# Autodesk Inventor assembly: Assembly_Cube_FluorescenceFilterSlider
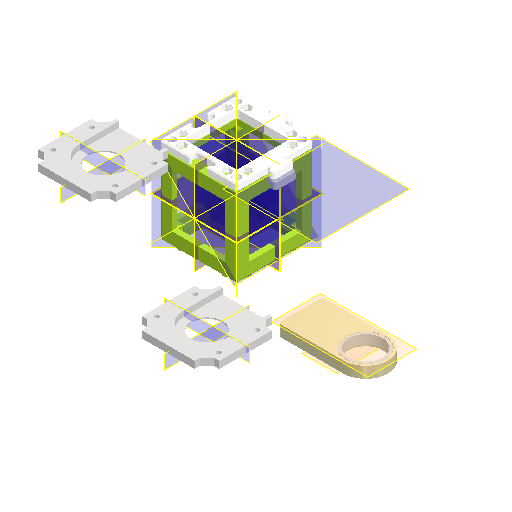
[picture p0: Inventor's stored thumbnail of the model, 512x512]
Saved by Autodesk Inventor 2025.1 (Build 291241020, 241B)
## iProperties
Created: 2023-11-21
Part Number: Assembly_Cube_FluorescenceFilterSlider
Document SubType Name: Assembly
Designer: diederichbenedict
Author: diederichbenedict
## Documents named in this file (5)
- C:\Users\diederichbenedict\Dropbox\Dokumente\Promotion\PROJECTS\openUC2-CAD\INVENTOR\Assembly_Cube_FluorescenceFilterSlider.iam
- C:\Users\diederichbenedict\Dropbox\Dokumente\Promotion\PROJECTS\openUC2-CAD\INVENTOR\20_Cube_Insert_Filterslide_25mm_v3.ipt
- C:\Users\diederichbenedict\Dropbox\Dokumente\Promotion\PROJECTS\openUC2-CAD\INVENTOR\10_Filteslide_25mm.ipt
- C:\Users\diederichbenedict\Dropbox\Dokumente\Promotion\PROJECTS\openUC2-CAD\INVENTOR\Assembly_Cube_empty_IM_v3.iam
- C:\Users\diederichbenedict\Dropbox\Dokumente\Promotion\PROJECTS\openUC2-CAD\INVENTOR\10_Filteslide_25mm_insert.ipt
## Components (5 placed, 4 different names)
1. 20_Cube_Insert_Filterslide_25mm_v3:1
2. 20_Cube_Insert_Filterslide_25mm_v3:2
3. 10_Filteslide_25mm:1 — Flush:1, Flush:2
4. Assembly_Cube_empty_IM_v3:1 [sub-assembly]
5. 10_Filteslide_25mm_insert:1 — Flush:1, Flush:2
## Relationships (2: Flush 2)
- Flush:1: 10_Filteslide_25mm:1 ↔ 10_Filteslide_25mm_insert:1
- Flush:2: 10_Filteslide_25mm:1 ↔ 10_Filteslide_25mm_insert:1
